# Autodesk Inventor assembly: mount_esc
Saved by Autodesk Inventor 2021 (Build 250183000, 183)
## iProperties
Created: 2021-01-23
Part Number: mount_esc
Document SubType Name: Assembly
Designer: User
Author: User
## Documents named in this file (3)
- D:\SynologyDrive\tcodev\tco-cad\mount_esc\mount_esc.iam
- D:\SynologyDrive\tcodev\tco-cad\mount_esc\mount_esc.ipt
- D:\SynologyDrive\tcodev\tco-cad\common\esc\esc.iam
## Components (2 placed, 2 different names)
1. mount_esc:1 — Mate:1, Mate:2, Mate:3
2. esc:1 [sub-assembly] — Mate:1, Mate:2, Mate:3
## Relationships (3: Mate 3)
- Mate:1: mount_esc:1 ↔ esc:1
- Mate:2 (0.5 mm): mount_esc:1 ↔ esc:1
- Mate:3 (0.25 mm): mount_esc:1 ↔ esc:1
